# Autodesk Inventor assembly: !arm
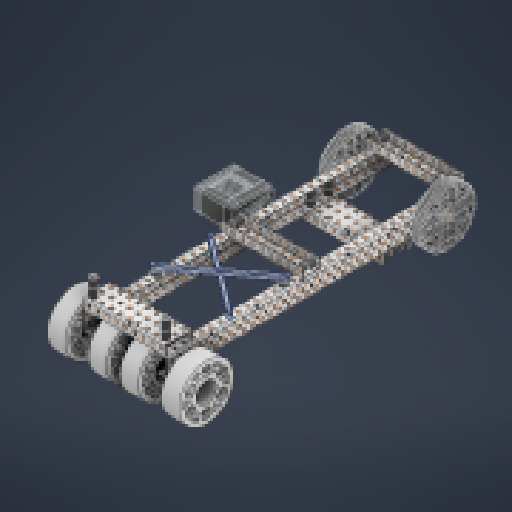
[picture p0: Inventor's stored thumbnail of the model, 512x512]
Saved by Autodesk Inventor 2024 (Build 280153000, 153)
## iProperties
Created: 2024-01-17
Part Number: !arm
Document SubType Name: Assembly
Designer: avere
Author: avere
## Documents named in this file (17)
- C:\Users\avere\Documents\rbp_cad\zoomba_v0.3\arm\!arm.iam
- C:\Users\avere\Documents\rbp_cad\VEX-CAD-Inventor-1.41\Motion\Gears\HS Gear\HS 72T Gear, No Insert.iam
- C:\Users\avere\Documents\rbp_cad\VEX-CAD-Inventor-1.41\Motion\Gears\HS Gear.iam
- C:\Users\avere\Documents\rbp_cad\VEX-CAD-Inventor-1.41\Structure\C Channel\Aluminum 1x2x1\Alu C 1x2x1x33.ipt
- C:\Users\avere\Documents\rbp_cad\VEX-CAD-Inventor-1.41\Motion\Shaft HS\HS Pillow Bearing Block.ipt
- C:\Users\avere\Documents\rbp_cad\VEX-CAD-Inventor-1.41\Motion\Wheels\Flex Wheels\3.000 Flex Wheel\3.000 30A 1.000.ipt
- C:\Users\avere\Documents\rbp_cad\VEX-CAD-Inventor-1.41\Motion\Wheels\Flex Wheels\3.000 Flex Wheel.ipt
- C:\Users\avere\Documents\rbp_cad\VEX-CAD-Inventor-1.41\Structure\C Channel\Aluminum 1x2x1\Alu C 1x2x1x9.ipt
- C:\Users\avere\Documents\rbp_cad\VEX-CAD-Inventor-1.41\Structure\C Channel\Aluminum 1x3x1\Alu C 1x3x1x9.ipt
- C:\Users\avere\Documents\rbp_cad\zoomba_v0.3\arm\custom_parts\xbrace_hs.ipt
- C:\Users\avere\Documents\rbp_cad\VEX-CAD-Inventor-1.41\Electronics\Motors with Screws\SteelM-StarS.iam
- C:\Users\avere\Documents\rbp_cad\VEX-CAD-Inventor-1.41\Electronics\Motors with Screws.iam
- C:\Users\avere\Documents\rbp_cad\VEX-CAD-Inventor-1.41\Motion\Spacers\Spacer Nylon .500 OD\NSpacer Black .500 OD x .250.ipt
- C:\Users\avere\Documents\rbp_cad\VEX-CAD-Inventor-1.41\Motion\Spacers\Spacer Nylon .500 OD.ipt
- C:\Users\avere\Documents\rbp_cad\VEX-CAD-Inventor-1.41\Motion\Spacers\Spacer Nylon .375 OD\NSpacer .375 OD x .500.ipt
- C:\Users\avere\Documents\rbp_cad\VEX-CAD-Inventor-1.41\Motion\Spacers\Spacer Nylon .375 OD.ipt
- C:\Users\avere\Documents\rbp_cad\VEX-CAD-Inventor-1.41\Motion\Spacers\Spacer Nylon .375 OD\NSpacer .375 OD x .375.ipt
## Components (45 placed, 11 different names)
1. HS 72T Gear, No Insert:1 [sub-assembly] — Insert:1, Mate:1
2. HS 72T Gear, No Insert:2 [sub-assembly] — Insert:5, Mate:4
3. Alu C 1x2x1x33:1 — Insert:1, Mate:1, Insert:3, Mate:2, Insert:12, Insert:15, Mate:11, Insert:17, Insert:32, Insert:33, Insert:42
4. HS Pillow Bearing Block:1 — Insert:2, Insert:9
5. 3.000 30A 1.000:1 — Insert:2
6. Alu C 1x2x1x9:1 — Insert:3, Mate:2, Insert:4, Mate:3, Insert:35, Insert:39
7. Alu C 1x2x1x33:2 — Insert:4, Mate:3, Insert:5, Mate:4, Insert:6, Mate:5, Mate:7, Mate:8, Insert:13, Mate:9, Insert:14, Mate:10, Insert:16, Insert:28, Insert:29
8. 3.000 30A 1.000:2 — Insert:7
9. HS Pillow Bearing Block:2 — Insert:6, Mate:5, Insert:7
10. 3.000 30A 1.000:3 — Insert:8
11. 3.000 30A 1.000:4 — Insert:8, Insert:9
12. Alu C 1x3x1x9:1 — Insert:14, Mate:10, Insert:26, Insert:27
13. xbrace_hs:1 — Insert:11, Mate:8
14. xbrace_hs:2 — Insert:11, Insert:12, Mate:7
15. SteelM-StarS:1 [sub-assembly] — Insert:13, Mate:9
16. Alu C 1x2x1x9:2 — Insert:15, Mate:11, Insert:40, Insert:41
17. NSpacer Black .500 OD x .250:1 — Insert:17
18. NSpacer Black .500 OD x .250:2 — Insert:16
19. NSpacer .375 OD x .500:1 — Insert:18
20. NSpacer .375 OD x .500:2 — Insert:18, Insert:19
21. NSpacer .375 OD x .375:3 — Insert:19, Insert:27
22. NSpacer .375 OD x .500:4
23. NSpacer .375 OD x .500:5
24. NSpacer .375 OD x .375:6 — Insert:26
25. NSpacer .375 OD x .500:8
26. NSpacer .375 OD x .375:9 — Insert:29
27. NSpacer .375 OD x .500:11
28. NSpacer .375 OD x .375:12 — Insert:28
29. NSpacer .375 OD x .500:13 — Insert:32
30. NSpacer .375 OD x .375:14
31. NSpacer .375 OD x .500:15 — Insert:33
32. NSpacer .375 OD x .375:16
33. NSpacer .375 OD x .500:17 — Insert:35
34. NSpacer .375 OD x .375:18
35. NSpacer .375 OD x .500:19 — Insert:41
36. NSpacer .375 OD x .375:20
37. NSpacer .375 OD x .500:21 — Insert:40
38. NSpacer .375 OD x .375:22
39. NSpacer .375 OD x .500:23 — Insert:39
40. NSpacer .375 OD x .375:24
41. Alu C 1x3x1x9:2 — Insert:42, Insert:43, Insert:44
42. NSpacer .375 OD x .500:25 — Insert:43, Insert:46
43. NSpacer .375 OD x .500:26 — Insert:44, Insert:45
44. NSpacer .375 OD x .500:27 — Insert:45
45. NSpacer .375 OD x .500:28 — Insert:46
## Relationships (53: Insert 43, Mate 10)
- Insert:1: HS 72T Gear, No Insert:1 ↔ Alu C 1x2x1x33:1
- Mate:1: HS 72T Gear, No Insert:1 ↔ Alu C 1x2x1x33:1
- Insert:2 (3.175 mm): HS Pillow Bearing Block:1 ↔ 3.000 30A 1.000:1
- Insert:3: Alu C 1x2x1x33:1 ↔ Alu C 1x2x1x9:1
- Mate:2: Alu C 1x2x1x33:1 ↔ Alu C 1x2x1x9:1
- Insert:4: Alu C 1x2x1x9:1 ↔ Alu C 1x2x1x33:2
- Mate:3: Alu C 1x2x1x9:1 ↔ Alu C 1x2x1x33:2
- Insert:5: HS 72T Gear, No Insert:2 ↔ Alu C 1x2x1x33:2
- Mate:4: HS 72T Gear, No Insert:2 ↔ Alu C 1x2x1x33:2
- Insert:6: Alu C 1x2x1x33:2 ↔ HS Pillow Bearing Block:2
- Mate:5: Alu C 1x2x1x33:2 ↔ HS Pillow Bearing Block:2
- Insert:7 (6.35 mm): 3.000 30A 1.000:2 ↔ HS Pillow Bearing Block:2
- Insert:8 (19.05 mm): 3.000 30A 1.000:3 ↔ 3.000 30A 1.000:4
- Insert:9 (15.875 mm): HS Pillow Bearing Block:1 ↔ 3.000 30A 1.000:4
- Insert:11: xbrace_hs:1 ↔ xbrace_hs:2
- Insert:12: Alu C 1x2x1x33:1 ↔ xbrace_hs:2
- Mate:7: Alu C 1x2x1x33:2 ↔ xbrace_hs:2
- Mate:8: Alu C 1x2x1x33:2 ↔ xbrace_hs:1
- Insert:13: Alu C 1x2x1x33:2 ↔ SteelM-StarS:1
- Mate:9: Alu C 1x2x1x33:2 ↔ SteelM-StarS:1
- Insert:14: Alu C 1x2x1x33:2 ↔ Alu C 1x3x1x9:1
- Mate:10: Alu C 1x2x1x33:2 ↔ Alu C 1x3x1x9:1
- Insert:15: Alu C 1x2x1x33:1 ↔ Alu C 1x2x1x9:2
- Mate:11: Alu C 1x2x1x33:1 ↔ Alu C 1x2x1x9:2
- Insert:16: Alu C 1x2x1x33:2 ↔ NSpacer Black .500 OD x .250:2
- Insert:17: Alu C 1x2x1x33:1 ↔ NSpacer Black .500 OD x .250:1
- Insert:18: NSpacer .375 OD x .500:1 ↔ NSpacer .375 OD x .500:2
- Insert:19: NSpacer .375 OD x .500:2 ↔ NSpacer .375 OD x .375:3
- [Insert]: NSpacer .375 OD x .500:4 ↔ NSpacer .375 OD x .500:5
- [Insert]: NSpacer .375 OD x .500:5 ↔ NSpacer .375 OD x .375:6
- [Insert]: NSpacer .375 OD x .500:8 ↔ NSpacer .375 OD x .375:9
- [Insert]: NSpacer .375 OD x .500:11 ↔ NSpacer .375 OD x .375:12
- Insert:26: Alu C 1x3x1x9:1 ↔ NSpacer .375 OD x .375:6
- Insert:27: Alu C 1x3x1x9:1 ↔ NSpacer .375 OD x .375:3
- Insert:28: Alu C 1x2x1x33:2 ↔ NSpacer .375 OD x .375:12
- Insert:29: Alu C 1x2x1x33:2 ↔ NSpacer .375 OD x .375:9
- [Insert]: NSpacer .375 OD x .500:13 ↔ NSpacer .375 OD x .375:14
- [Insert]: NSpacer .375 OD x .500:15 ↔ NSpacer .375 OD x .375:16
- Insert:32: Alu C 1x2x1x33:1 ↔ NSpacer .375 OD x .500:13
- Insert:33: Alu C 1x2x1x33:1 ↔ NSpacer .375 OD x .500:15
- [Insert]: NSpacer .375 OD x .500:17 ↔ NSpacer .375 OD x .375:18
- Insert:35: Alu C 1x2x1x9:1 ↔ NSpacer .375 OD x .500:17
- [Insert]: NSpacer .375 OD x .500:19 ↔ NSpacer .375 OD x .375:20
- [Insert]: NSpacer .375 OD x .500:21 ↔ NSpacer .375 OD x .375:22
- [Insert]: NSpacer .375 OD x .500:23 ↔ NSpacer .375 OD x .375:24
- Insert:39: Alu C 1x2x1x9:1 ↔ NSpacer .375 OD x .500:23
- Insert:40: Alu C 1x2x1x9:2 ↔ NSpacer .375 OD x .500:21
- Insert:41: Alu C 1x2x1x9:2 ↔ NSpacer .375 OD x .500:19
- Insert:42 (15.0812 mm): Alu C 1x2x1x33:1 ↔ Alu C 1x3x1x9:2
- Insert:43: Alu C 1x3x1x9:2 ↔ NSpacer .375 OD x .500:25
- Insert:44: Alu C 1x3x1x9:2 ↔ NSpacer .375 OD x .500:26
- Insert:45: NSpacer .375 OD x .500:26 ↔ NSpacer .375 OD x .500:27
- Insert:46: NSpacer .375 OD x .500:25 ↔ NSpacer .375 OD x .500:28
## Named parameters: d35_d33 = 0 mm, d36_d34 = 0 mm, d38_d34 = 0 mm, d40_d34 = 0 mm, d45_d40_d34 = 0 mm, d46_d40_d34 = 0 mm, d49_d40_d34 = 0 mm, d51_d40_d34 = 0 mm, d52_d40_d34 = 0 mm, d53_d40_d34 = 0 mm
